# Autodesk Inventor assembly: motor
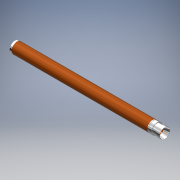
[picture p0: Inventor's stored thumbnail of the model, 180x180]
Saved by Autodesk Inventor 2017 SP1 (Build 210196100, 196)
## iProperties
Created: 2016-10-29
Part Number: motor
Document SubType Name: Assembly
Designer: cflannery
Author: cflannery
## Documents named in this file (7)
- D:\Triton_Rocket_Club\Propulsion\Launches\8-inch-flight\Design\CAD\Vehicle\Structures\motor.iam
- D:\Triton_Rocket_Club\Propulsion\Launches\8-inch-flight\Design\CAD\Vehicle\Structures\casting_tube.ipt
- D:\Triton_Rocket_Club\Propulsion\Launches\8-inch-flight\Design\CAD\Vehicle\Structures\grain.ipt
- D:\Triton_Rocket_Club\Propulsion\Launches\8-inch-flight\Design\CAD\Vehicle\Structures\phenolic_liner.ipt
- D:\Triton_Rocket_Club\Propulsion\Launches\8-inch-flight\Design\CAD\Vehicle\Structures\thermal_barrier.ipt
- D:\Triton_Rocket_Club\Propulsion\Launches\8-inch-flight\Design\CAD\Vehicle\Nozzle\trunk\nozzle.iam
- D:\Triton_Rocket_Club\Propulsion\Launches\8-inch-flight\Design\CAD\Vehicle\Nozzle\trunk\motor_bulkhead.ipt
## Components (16 placed, 6 different names)
1. casting_tube:1 — Mate:5, Flush:5, Mate:8, Mate:9, Mate:10, Mate:11, Mate:15, Mate:16
2. grain:1 — Mate:5, Flush:5
3. phenolic_liner:1 — Flush:7, Mate:18, Mate:19, Mate:20, Mate:22, Mate:23
4. casting_tube:2 — Mate:3, Flush:2, Mate:9, Mate:14, Mate:15
5. grain:2 — Mate:3, Flush:2
6. casting_tube:3 — Mate:2, Flush:3, Mate:10, Mate:12, Mate:16, Mate:17
7. grain:3 — Mate:2, Flush:3
8. casting_tube:4 — Mate:1, Flush:1, Mate:12, Mate:13
9. grain:4 — Mate:1, Flush:1, Mate:21
10. casting_tube:5 — Mate:4, Flush:6, Mate:11, Mate:13, Mate:14
11. grain:5 — Mate:4, Flush:6
12. casting_tube:6 — Mate:6, Flush:4, Mate:8, Mate:17, Flush:7, Mate:18
13. grain:6 — Mate:6, Flush:4
14. thermal_barrier:1 — Mate:19, Mate:20, Mate:24, Mate:25
15. nozzle:1 [sub-assembly] — Mate:21, Mate:22
16. motor_bulkhead:1 — Mate:23, Mate:24, Mate:25
## Relationships (31: Mate 24, Flush 7)
- Mate:1: casting_tube:4 ↔ grain:4
- Flush:1 (12.7 mm): casting_tube:4 ↔ grain:4
- Mate:2: casting_tube:3 ↔ grain:3
- Mate:3: casting_tube:2 ↔ grain:2
- Mate:4: casting_tube:5 ↔ grain:5
- Mate:5: casting_tube:1 ↔ grain:1
- Mate:6: casting_tube:6 ↔ grain:6
- Flush:2 (12.7 mm): casting_tube:2 ↔ grain:2
- Flush:3 (12.7 mm): casting_tube:3 ↔ grain:3
- Flush:4 (12.7 mm): casting_tube:6 ↔ grain:6
- Flush:5 (12.7 mm): casting_tube:1 ↔ grain:1
- Flush:6 (12.7 mm): casting_tube:5 ↔ grain:5
- Mate:8: casting_tube:1 ↔ casting_tube:6
- Mate:9: casting_tube:1 ↔ casting_tube:2
- Mate:10: casting_tube:1 ↔ casting_tube:3
- Mate:11: casting_tube:1 ↔ casting_tube:5
- Mate:12: casting_tube:3 ↔ casting_tube:4
- Mate:13: casting_tube:4 ↔ casting_tube:5
- Mate:14: casting_tube:2 ↔ casting_tube:5
- Mate:15: casting_tube:1 ↔ casting_tube:2
- Mate:16: casting_tube:1 ↔ casting_tube:3
- Mate:17: casting_tube:3 ↔ casting_tube:6
- Flush:7 (12.7 mm): phenolic_liner:1 ↔ casting_tube:6
- Mate:18: phenolic_liner:1 ↔ casting_tube:6
- Mate:19: phenolic_liner:1 ↔ thermal_barrier:1
- Mate:20: phenolic_liner:1 ↔ thermal_barrier:1
- Mate:21: grain:4 ↔ nozzle:1
- Mate:22: phenolic_liner:1 ↔ nozzle:1
- Mate:23: phenolic_liner:1 ↔ motor_bulkhead:1
- Mate:24: thermal_barrier:1 ↔ motor_bulkhead:1
- Mate:25: thermal_barrier:1 ↔ motor_bulkhead:1
